# Autodesk Inventor assembly: Фильтр D1200
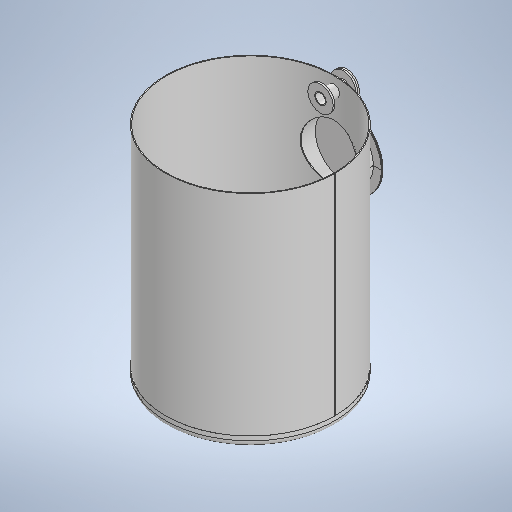
[picture p0: Inventor's stored thumbnail of the model, 512x512]
Saved by Autodesk Inventor 2025 (Build 290162010, 162A)
## iProperties
Created: 2025-02-13
Part Number: Фильтр D1200
Document SubType Name: Assembly
Designer: pokla
Author: pokla
## Documents named in this file (10)
- C:\Users\pokla\Desktop\Работа Акватроник\Фильтры напорные\D1200\Фильтр D1200.iam
- C:\Users\pokla\Desktop\Работа Акватроник\Фильтры напорные\D1200\Заглушка ревиз. окна фильтра D1200.ipt
- C:\Users\pokla\Desktop\Работа Акватроник\Фильтры напорные\D1200\Заглушка фланца трубы подключения фильтра D1200.ipt
- C:\Users\pokla\Desktop\Работа Акватроник\Фильтры напорные\D1200\Кольцо заглушки ревиз. окна фильтра D1200.ipt
- C:\Users\pokla\Desktop\Работа Акватроник\Фильтры напорные\D1200\Размеры D1200.ipt
- C:\Users\pokla\Desktop\Работа Акватроник\Фильтры напорные\D1200\Ревиз. окно фильтра D1200.ipt
- C:\Users\pokla\Desktop\Работа Акватроник\Фильтры напорные\D1200\Стенка фильтра D1200.ipt
- C:\Users\pokla\Desktop\Работа Акватроник\Фильтры напорные\D1200\Труба подключения фильтра D1200.ipt
- C:\Users\pokla\Desktop\Работа Акватроник\Фильтры напорные\D1200\Фланец трубы подключения фильтра D1200.ipt
- C:\Users\pokla\Desktop\Работа Акватроник\Фильтры напорные\D1200\Сферическое дно D1200.ipt
## Components (15 placed, 9 different names)
1. Заглушка ревиз. окна фильтра D1200:1 — Rigid:12
2. Заглушка фланца трубы подключения фильтра D1200:1 — Rigid:4
3. Кольцо заглушки ревиз. окна фильтра D1200:1 — Rigid:1, Rigid:11
4. Размеры D1200:1
5. Ревиз. окно фильтра D1200:1 — Rigid:10, Rigid:11, Rigid:12
6. Стенка фильтра D1200:1 — Rigid:5, Rigid:9, Rigid:10, Rigid:13
7. Труба подключения фильтра D1200:1 — Rigid:2, Rigid:3, Rigid:5
8. Фланец трубы подключения фильтра D1200:1 — Rigid:2, Rigid:4
9. Кольцо заглушки ревиз. окна фильтра D1200:2 — Rigid:1
10. Фланец трубы подключения фильтра D1200:2 — Rigid:3
11. Заглушка фланца трубы подключения фильтра D1200:2
12. Труба подключения фильтра D1200:2 — Rigid:9
13. Фланец трубы подключения фильтра D1200:3
14. Фланец трубы подключения фильтра D1200:4
15. Сферическое дно D1200:1 — Rigid:13
## Relationships (13: WeldJoint 13)
- Rigid:1 [WeldJoint]: Кольцо заглушки ревиз. окна фильтра D1200:1 ↔ Кольцо заглушки ревиз. окна фильтра D1200:2
- Rigid:2 [WeldJoint]: Труба подключения фильтра D1200:1 ↔ Фланец трубы подключения фильтра D1200:1
- Rigid:3 [WeldJoint]: Труба подключения фильтра D1200:1 ↔ Фланец трубы подключения фильтра D1200:2
- Rigid:4 [WeldJoint]: Заглушка фланца трубы подключения фильтра D1200:1 ↔ Фланец трубы подключения фильтра D1200:1
- Rigid:5 [WeldJoint] (97 mm): Стенка фильтра D1200:1 ↔ Труба подключения фильтра D1200:1
- [WeldJoint]: Труба подключения фильтра D1200:2 ↔ Фланец трубы подключения фильтра D1200:3
- [WeldJoint]: Труба подключения фильтра D1200:2 ↔ Фланец трубы подключения фильтра D1200:4
- [WeldJoint]: Заглушка фланца трубы подключения фильтра D1200:2 ↔ Фланец трубы подключения фильтра D1200:3
- Rigid:9 [WeldJoint] (97 mm): Стенка фильтра D1200:1 ↔ Труба подключения фильтра D1200:2
- Rigid:10 [WeldJoint] (66 mm): Ревиз. окно фильтра D1200:1 ↔ Стенка фильтра D1200:1
- Rigid:11 [WeldJoint]: Кольцо заглушки ревиз. окна фильтра D1200:1 ↔ Ревиз. окно фильтра D1200:1
- Rigid:12 [WeldJoint]: Заглушка ревиз. окна фильтра D1200:1 ↔ Ревиз. окно фильтра D1200:1
- Rigid:13 [WeldJoint]: Стенка фильтра D1200:1 ↔ Сферическое дно D1200:1
## Named parameters: d5_d3 = 0 mm, d6_d1 = 0 mm, d7_d2 = 0 mm
